# Autodesk Inventor assembly: Montagem_corpo_menor
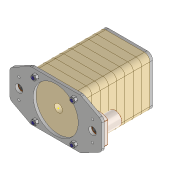
[picture p0: Inventor's stored thumbnail of the model, 180x180]
Saved by Autodesk Inventor 2020 (Build 240168000, 168)
## iProperties
Created: 2022-07-20
Part Number: Montagem_corpo_menor
Document SubType Name: Assembly
Designer: gabri
Author: gabri
## Documents named in this file (8)
- C:\Users\gabri\OneDrive\Área de Trabalho\Calorimetro 2022\Calorimetro github\Inventor\Montagem_corpo_menor.iam
- C:\Users\gabri\OneDrive\Área de Trabalho\Calorimetro 2022\Calorimetro github\Inventor\Suporte_inferior_menor.ipt
- C:\Users\gabri\OneDrive\Área de Trabalho\Calorimetro 2022\Calorimetro github\Inventor\corpo_2_menor.ipt
- C:\Users\gabri\OneDrive\Área de Trabalho\Calorimetro 2022\Calorimetro github\Inventor\corpo_1_menor.ipt
- C:\Users\gabri\OneDrive\Área de Trabalho\Calorimetro 2022\Calorimetro github\Inventor\Suporte_superior_menor.ipt
- C:\Users\gabri\OneDrive\Área de Trabalho\Calorimetro 2022\Calorimetro github\Inventor\tampa.ipt
- C:\Users\gabri\OneDrive\Área de Trabalho\Calorimetro 2022\Calorimetro github\Inventor\LMH10UUx29.ipt
- C:\Users\gabri\OneDrive\Área de Trabalho\Calorimetro 2022\Calorimetro github\Inventor\porcaM4.ipt
## Components (17 placed, 7 different names)
1. Suporte_inferior_menor:1 — Coincidência:1, Coincidência:2, Coincidência:11, Coincidência:12, Coincidência:13, Coincidência:14, Coincidência:15, Coincidência:16, Coincidência:17, Coincidência:18, Coincidência:19, Coincidência:20, Coincidência:21, Coincidência:22, Coincidência:23, Coincidência:24
2. corpo_1_menor:1 — Coincidência:1, Coincidência:2, Coincidência:3, Coincidência:4, Coincidência:6
3. Suporte_superior_menor:1 — Coincidência:7, Coincidência:8, Coincidência:10
4. tampa:1 — Coincidência:9, Coincidência:10
5. LMH10UUx29:1 — Coincidência:14, Coincidência:15, Coincidência:16
6. LMH10UUx29:2 — Coincidência:11, Coincidência:12, Coincidência:13
7. porcaM4:1 — Coincidência:18, Coincidência:22
8. porcaM4:2 — Coincidência:17, Coincidência:24
9. porcaM4:3 — Coincidência:19, Coincidência:23
10. porcaM4:4 — Coincidência:20, Coincidência:21
11. corpo_2_menor:1 — Coincidência:3, Coincidência:4
12. corpo_2_menor:2
13. corpo_2_menor:3
14. corpo_2_menor:4 — Coincidência:5
15. corpo_1_menor:2 — Coincidência:5, Coincidência:6
16. corpo_1_menor:3
17. corpo_1_menor:4 — Coincidência:7, Coincidência:8, Coincidência:9
## Component patterns: (4 elements, first: corpo_2_menor:1), (3 elements, first: corpo_1_menor:2)
## Relationships (24: Mate 24)
- Coincidência:1 [Mate]: Suporte_inferior_menor:1 ↔ corpo_1_menor:1
- Coincidência:2 [Mate]: Suporte_inferior_menor:1 ↔ corpo_1_menor:1
- Coincidência:3 [Mate]: corpo_1_menor:1 ↔ corpo_2_menor:1
- Coincidência:4 [Mate]: corpo_1_menor:1 ↔ corpo_2_menor:1
- Coincidência:5 [Mate]: corpo_2_menor:4 ↔ corpo_1_menor:2
- Coincidência:6 [Mate]: corpo_1_menor:1 ↔ corpo_1_menor:2
- Coincidência:7 [Mate]: Suporte_superior_menor:1 ↔ corpo_1_menor:4
- Coincidência:8 [Mate]: Suporte_superior_menor:1 ↔ corpo_1_menor:4
- Coincidência:9 [Mate]: tampa:1 ↔ corpo_1_menor:4
- Coincidência:10 [Mate]: Suporte_superior_menor:1 ↔ tampa:1
- Coincidência:11 [Mate]: Suporte_inferior_menor:1 ↔ LMH10UUx29:2
- Coincidência:12 [Mate]: Suporte_inferior_menor:1 ↔ LMH10UUx29:2
- Coincidência:13 [Mate]: Suporte_inferior_menor:1 ↔ LMH10UUx29:2
- Coincidência:14 [Mate]: Suporte_inferior_menor:1 ↔ LMH10UUx29:1
- Coincidência:15 [Mate]: Suporte_inferior_menor:1 ↔ LMH10UUx29:1
- Coincidência:16 [Mate]: Suporte_inferior_menor:1 ↔ LMH10UUx29:1
- Coincidência:17 [Mate]: Suporte_inferior_menor:1 ↔ porcaM4:2
- Coincidência:18 [Mate]: Suporte_inferior_menor:1 ↔ porcaM4:1
- Coincidência:19 [Mate]: Suporte_inferior_menor:1 ↔ porcaM4:3
- Coincidência:20 [Mate]: Suporte_inferior_menor:1 ↔ porcaM4:4
- Coincidência:21 [Mate]: Suporte_inferior_menor:1 ↔ porcaM4:4
- Coincidência:22 [Mate]: Suporte_inferior_menor:1 ↔ porcaM4:1
- Coincidência:23 [Mate]: Suporte_inferior_menor:1 ↔ porcaM4:3
- Coincidência:24 [Mate]: Suporte_inferior_menor:1 ↔ porcaM4:2
